# Autodesk Inventor assembly: ArmadoNewtonCart
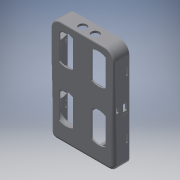
[picture p0: Inventor's stored thumbnail of the model, 180x180]
Saved by Autodesk Inventor 2019 (Build 230136000, 136)
## iProperties
Created: 2020-10-10
Part Number: ArmadoNewtonCart
Document SubType Name: Assembly
Designer: peter
Author: peter
## Documents named in this file (3)
- C:\Users\ThinkPad\Documents\GitHub\Newton-Cart\3D Platform design\ArmadoNewtonCart.iam
- C:\Users\ThinkPad\Documents\GitHub\Newton-Cart\3D Platform design\Carcasa1.ipt
- C:\Users\ThinkPad\Documents\GitHub\Newton-Cart\3D Platform design\garracomp3.ipt
## Components (5 placed, 2 different names)
1. Carcasa1:1 — Mate:1, Mate:2, Mate:3, Mate:4, Mate:5, Mate:6, Mate:7, Mate:8, Mate:9, Mate:10, Mate:11, Mate:12, Mate:13, Mate:14
2. garracomp3:1 — Mate:1, Mate:2, Mate:3, Mate:13
3. garracomp3:2 — Mate:6, Mate:7, Mate:11
4. garracomp3:3 — Mate:8, Mate:9, Mate:10
5. garracomp3:4 — Mate:4, Mate:5, Mate:12, Mate:14
## Relationships (14: Mate 14)
- Mate:1: Carcasa1:1 ↔ garracomp3:1
- Mate:2: Carcasa1:1 ↔ garracomp3:1
- Mate:3: Carcasa1:1 ↔ garracomp3:1
- Mate:4: Carcasa1:1 ↔ garracomp3:4
- Mate:5: Carcasa1:1 ↔ garracomp3:4
- Mate:6: Carcasa1:1 ↔ garracomp3:2
- Mate:7: Carcasa1:1 ↔ garracomp3:2
- Mate:8: Carcasa1:1 ↔ garracomp3:3
- Mate:9: Carcasa1:1 ↔ garracomp3:3
- Mate:10: Carcasa1:1 ↔ garracomp3:3
- Mate:11: Carcasa1:1 ↔ garracomp3:2
- Mate:12: Carcasa1:1 ↔ garracomp3:4
- Mate:13: Carcasa1:1 ↔ garracomp3:1
- Mate:14: Carcasa1:1 ↔ garracomp3:4
